# Autodesk Inventor assembly: assemmbly skyhunter
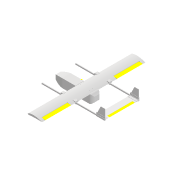
[picture p0: Inventor's stored thumbnail of the model, 180x180]
Saved by Autodesk Inventor 2020 (Build 240168000, 168)
## iProperties
Created: 2020-03-09
Part Number: assemmbly skyhunter
Document SubType Name: Assembly
Designer: alifhabib
Author: alifhabib
## Documents named in this file (11)
- D:\PENS\Projek Akhir\skyhunter desain\tiap part assembly\assemmbly skyhunter.iam
- D:\PENS\Projek Akhir\skyhunter desain\tiap part assembly\wing.ipt
- D:\PENS\Projek Akhir\skyhunter desain\tiap part assembly\elevatotr.ipt
- D:\PENS\Projek Akhir\skyhunter desain\body\tiap part\penghubung rudder elevator.ipt
- D:\PENS\Projek Akhir\skyhunter desain\body\tiap part\penghubung rudder elevato kananr.ipt
- D:\PENS\Projek Akhir\skyhunter desain\tiap part assembly\rudder.ipt
- D:\PENS\Projek Akhir\skyhunter desain\tiap part assembly\batang.ipt
- D:\PENS\Projek Akhir\skyhunter desain\body\tiap part\hub sayap belakang.ipt
- D:\PENS\Projek Akhir\skyhunter desain\body\tiap part\hub sayap belakang_MIR.ipt
- D:\PENS\Projek Akhir\skyhunter desain\body\tiap part\hub sayap depan.ipt
- D:\PENS\Projek Akhir\skyhunter desain\tiap part assembly\body.ipt
## Components (13 placed, 10 different names)
1. wing:1
2. elevatotr:1 — Mate:5, Mate:6, Mate:7, Mate:8, Mate:9, Mate:10
3. penghubung rudder elevato kananr:1 — Mate:5, Mate:7, Mate:10, Mate:14, Mate:15, Mate:16, Mate:19, Mate:20, Symmetry:1
4. penghubung rudder elevator:1 — Mate:6, Mate:8, Mate:9, Mate:11, Mate:12, Mate:13, Mate:17, Mate:18, Symmetry:1
5. rudder:1 — Mate:11, Mate:12, Mate:13
6. rudder:2 — Mate:14, Mate:15, Mate:16
7. batang:1 — Mate:17, Mate:18, Mate:21, Mate:22
8. batang:2 — Mate:19, Mate:20
9. hub sayap belakang:1 — Mate:21, Mate:22
10. hub sayap belakang_MIR:1
11. hub sayap depan:1
12. hub sayap depan:2
13. body:1
## Relationships (19: Mate 18, Symmetry 1)
- Mate:5: elevatotr:1 ↔ penghubung rudder elevato kananr:1
- Mate:6: elevatotr:1 ↔ penghubung rudder elevator:1
- Mate:7: elevatotr:1 ↔ penghubung rudder elevato kananr:1
- Mate:8: elevatotr:1 ↔ penghubung rudder elevator:1
- Mate:9: elevatotr:1 ↔ penghubung rudder elevator:1
- Mate:10: elevatotr:1 ↔ penghubung rudder elevato kananr:1
- Mate:11: penghubung rudder elevator:1 ↔ rudder:1
- Mate:12: penghubung rudder elevator:1 ↔ rudder:1
- Mate:13: penghubung rudder elevator:1 ↔ rudder:1
- Mate:14: penghubung rudder elevato kananr:1 ↔ rudder:2
- Mate:15: penghubung rudder elevato kananr:1 ↔ rudder:2
- Mate:16: penghubung rudder elevato kananr:1 ↔ rudder:2
- Mate:17: penghubung rudder elevator:1 ↔ batang:1
- Mate:18: penghubung rudder elevator:1 ↔ batang:1
- Mate:19: penghubung rudder elevato kananr:1 ↔ batang:2
- Mate:20: penghubung rudder elevato kananr:1 ↔ batang:2
- Mate:21: batang:1 ↔ hub sayap belakang:1
- Mate:22: batang:1 ↔ hub sayap belakang:1
- Symmetry:1: penghubung rudder elevato kananr:1 ↔ penghubung rudder elevator:1
